# Autodesk Inventor assembly: Servo and Frame
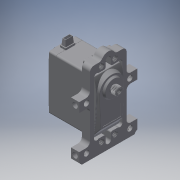
[picture p0: Inventor's stored thumbnail of the model, 180x180]
Saved by Autodesk Inventor 2019 (Build 230136000, 136)
## iProperties
Created: 2018-11-18
Part Number: Servo and Frame
Document SubType Name: Assembly
Designer: Ashley
Author: Ashley
## Documents named in this file (3)
- C:\Users\Ashley\Desktop\repositories\design\inventor\Imported Components\goBilda\Servo and Frame.iam
- C:\Users\Ashley\Desktop\repositories\design\inventor\Imported Components\goBilda\goBildaServo.ipt
- C:\Users\Ashley\Desktop\repositories\design\inventor\Imported Components\goBilda\1802SeriesServoFrame.ipt
## Components (2 placed, 2 different names)
1. goBildaServo:1 — Mate:1
2. 1802SeriesServoFrame:1 — Mate:1
## Relationships (1: Mate 1)
- Mate:1: goBildaServo:1 ↔ 1802SeriesServoFrame:1
